# Autodesk Inventor assembly: Sideassembly
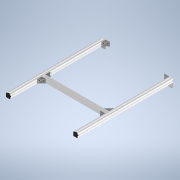
[picture p0: Inventor's stored thumbnail of the model, 180x180]
Saved by Autodesk Inventor 2020.2 (Build 242310000, 310)
## iProperties
Created: 2020-07-25
Part Number: Sideassembly
Document SubType Name: Assembly
Designer: JK
Author: JK
## Documents named in this file (3)
- C:\Users\JK\Documents\Inventor\Mesa\Sideassembly.iam
- C:\Users\JK\Documents\Inventor\Mesa\Legassembly.iam
- C:\Users\JK\Documents\Inventor\Mesa\Legstretcher.iam
## Components (3 placed, 2 different names)
1. Legassembly:1 [sub-assembly] — Mate:1, Flush:1, Flush:3
2. Legassembly:2 [sub-assembly] — Mate:2, Flush:2, Flush:3, Flush:4
3. Legstretcher:1 [sub-assembly] — Mate:1, Flush:1, Mate:2, Flush:2, Flush:4
## Relationships (6: Flush 4, Mate 2)
- Mate:1: Legassembly:1 ↔ Legstretcher:1
- Flush:1 (0.5 mm): Legassembly:1 ↔ Legstretcher:1
- Mate:2: Legassembly:2 ↔ Legstretcher:1
- Flush:2 (0.5 mm): Legassembly:2 ↔ Legstretcher:1
- Flush:3: Legassembly:1 ↔ Legassembly:2
- Flush:4 (250 mm): Legassembly:2 ↔ Legstretcher:1
